# Autodesk Inventor assembly: Mechunam base 1.10
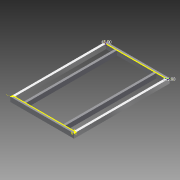
[picture p0: Inventor's stored thumbnail of the model, 180x180]
Saved by Autodesk Inventor 2015 (Build 190159000, 159)
## iProperties
Created: 2015-01-11
Part Number: Mechunam base 1.10
Document SubType Name: Weldment
Designer: chapale16
Weld Material: Welded Aluminum-6061
Author: chapale16
## Documents named in this file (7)
- H:\Mechunam base 1.10.iam
- H:\42in 2x1 boxbeam.ipt
- H:\40in 2x1 boxbeam.ipt
- H:\28in 1x2.ipt
- H:\40in 2x1 boxbeam_MIR_MIR.ipt
- H:\28in 1x2_MIR1_MIR.ipt
- H:\42in 2x1 boxbeam_MIR1_MIR.ipt
## Components (6 placed, 6 different names)
1. 40in 2x1 boxbeam:4 — Mate:3, Mate:4
2. 28in 1x2:1 — Mate:1, Mate:2, Mate:4
3. 42in 2x1 boxbeam:2 — Mate:1, Mate:2, Mate:3, Mate:17, Mate:18
4. 40in 2x1 boxbeam_MIR_MIR:1 — Mate:13, Mate:14
5. 28in 1x2_MIR1_MIR:1 — Mate:13, Mate:15, Mate:16, Mate:17, Mate:18
6. 42in 2x1 boxbeam_MIR1_MIR:1 — Mate:14, Mate:15, Mate:16
## Relationships (10: Mate 10)
- Mate:1: 28in 1x2:1 ↔ 42in 2x1 boxbeam:2
- Mate:2: 28in 1x2:1 ↔ 42in 2x1 boxbeam:2
- Mate:3 (98.425 mm): 40in 2x1 boxbeam:4 ↔ 42in 2x1 boxbeam:2
- Mate:4: 40in 2x1 boxbeam:4 ↔ 28in 1x2:1
- Mate:13: 40in 2x1 boxbeam_MIR_MIR:1 ↔ 28in 1x2_MIR1_MIR:1
- Mate:14 (98.425 mm): 40in 2x1 boxbeam_MIR_MIR:1 ↔ 42in 2x1 boxbeam_MIR1_MIR:1
- Mate:15: 28in 1x2_MIR1_MIR:1 ↔ 42in 2x1 boxbeam_MIR1_MIR:1
- Mate:16: 28in 1x2_MIR1_MIR:1 ↔ 42in 2x1 boxbeam_MIR1_MIR:1
- Mate:17: 42in 2x1 boxbeam:2 ↔ 28in 1x2_MIR1_MIR:1
- Mate:18: 42in 2x1 boxbeam:2 ↔ 28in 1x2_MIR1_MIR:1
